# Autodesk Inventor assembly: CC
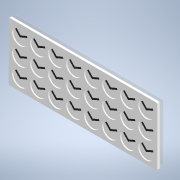
[picture p0: Inventor's stored thumbnail of the model, 180x180]
Saved by Autodesk Inventor 2020 (Build 240168000, 168)
## iProperties
Created: 2019-07-03
Part Number: CC
Document SubType Name: Assembly
Designer: andwh
Author: andwh
## Documents named in this file (6)
- C:\Users\andwh\Documents\Projects\Clock Clock\CC.iam
- C:\Users\andwh\Documents\Projects\Clock Clock\CC-topPlate.ipt
- C:\Users\andwh\Documents\Projects\Clock Clock\Parts\94459A140_BRASS HEAT-SET INSERT FOR PLASTIC.ipt
- C:\Users\andwh\Documents\Projects\Clock Clock\PCB\Clock Board V2\Clock Board V2.iam
- C:\Users\andwh\Documents\Projects\Clock Clock\CC-bottomStand.ipt
- C:\Users\andwh\Documents\Projects\Clock Clock\CC-bottomPlate.ipt
## Components (126 placed, 5 different names)
1. CC-topPlate:1 — Insert:1, Insert:2, Mate:1
2. CC-bottomPlate:1 — Insert:5, Insert:6
3. Clock Board V2:1 [sub-assembly] — Insert:2, Mate:1
4. Clock Board V2:2 [sub-assembly]
5. Clock Board V2:3 [sub-assembly]
6. Clock Board V2:4 [sub-assembly]
7. Clock Board V2:5 [sub-assembly]
8. Clock Board V2:6 [sub-assembly]
9. Clock Board V2:7 [sub-assembly]
10. Clock Board V2:8 [sub-assembly]
11. Clock Board V2:9 [sub-assembly]
12. Clock Board V2:10 [sub-assembly]
13. Clock Board V2:11 [sub-assembly]
14. Clock Board V2:12 [sub-assembly]
15. Clock Board V2:13 [sub-assembly]
16. Clock Board V2:14 [sub-assembly]
17. Clock Board V2:15 [sub-assembly]
18. Clock Board V2:16 [sub-assembly]
19. Clock Board V2:17 [sub-assembly]
20. Clock Board V2:18 [sub-assembly]
21. Clock Board V2:19 [sub-assembly] — Insert:4
22. Clock Board V2:20 [sub-assembly]
23. Clock Board V2:21 [sub-assembly]
24. Clock Board V2:22 [sub-assembly] — Insert:3
25. Clock Board V2:23 [sub-assembly]
26. Clock Board V2:24 [sub-assembly] — Insert:5, Insert:6
27. CC-bottomStand:1 — Insert:3, Insert:4
28. CC-bottomStand:2
29. CC-bottomStand:3
30. CC-bottomStand:4
31. 94459A140_BRASS HEAT-SET INSERT FOR PLASTIC:1 — Insert:1
32. 94459A140_BRASS HEAT-SET INSERT FOR PLASTIC:2
33. 94459A140_BRASS HEAT-SET INSERT FOR PLASTIC:3
34. 94459A140_BRASS HEAT-SET INSERT FOR PLASTIC:4
35. 94459A140_BRASS HEAT-SET INSERT FOR PLASTIC:5
36. 94459A140_BRASS HEAT-SET INSERT FOR PLASTIC:6
37. 94459A140_BRASS HEAT-SET INSERT FOR PLASTIC:7
38. 94459A140_BRASS HEAT-SET INSERT FOR PLASTIC:8
39. 94459A140_BRASS HEAT-SET INSERT FOR PLASTIC:9
40. 94459A140_BRASS HEAT-SET INSERT FOR PLASTIC:10
41. 94459A140_BRASS HEAT-SET INSERT FOR PLASTIC:11
42. 94459A140_BRASS HEAT-SET INSERT FOR PLASTIC:12
43. 94459A140_BRASS HEAT-SET INSERT FOR PLASTIC:13
44. 94459A140_BRASS HEAT-SET INSERT FOR PLASTIC:14
45. 94459A140_BRASS HEAT-SET INSERT FOR PLASTIC:15
46. 94459A140_BRASS HEAT-SET INSERT FOR PLASTIC:16
47. 94459A140_BRASS HEAT-SET INSERT FOR PLASTIC:17
48. 94459A140_BRASS HEAT-SET INSERT FOR PLASTIC:18
49. 94459A140_BRASS HEAT-SET INSERT FOR PLASTIC:19
50. 94459A140_BRASS HEAT-SET INSERT FOR PLASTIC:20
51. 94459A140_BRASS HEAT-SET INSERT FOR PLASTIC:21
52. 94459A140_BRASS HEAT-SET INSERT FOR PLASTIC:22
53. 94459A140_BRASS HEAT-SET INSERT FOR PLASTIC:23
54. 94459A140_BRASS HEAT-SET INSERT FOR PLASTIC:24
55. 94459A140_BRASS HEAT-SET INSERT FOR PLASTIC:25
56. 94459A140_BRASS HEAT-SET INSERT FOR PLASTIC:26
57. 94459A140_BRASS HEAT-SET INSERT FOR PLASTIC:27
58. 94459A140_BRASS HEAT-SET INSERT FOR PLASTIC:28
59. 94459A140_BRASS HEAT-SET INSERT FOR PLASTIC:29
60. 94459A140_BRASS HEAT-SET INSERT FOR PLASTIC:30
61. 94459A140_BRASS HEAT-SET INSERT FOR PLASTIC:31
62. 94459A140_BRASS HEAT-SET INSERT FOR PLASTIC:32
63. 94459A140_BRASS HEAT-SET INSERT FOR PLASTIC:33
64. 94459A140_BRASS HEAT-SET INSERT FOR PLASTIC:34
65. 94459A140_BRASS HEAT-SET INSERT FOR PLASTIC:35
66. 94459A140_BRASS HEAT-SET INSERT FOR PLASTIC:36
67. 94459A140_BRASS HEAT-SET INSERT FOR PLASTIC:37
68. 94459A140_BRASS HEAT-SET INSERT FOR PLASTIC:38
69. 94459A140_BRASS HEAT-SET INSERT FOR PLASTIC:39
70. 94459A140_BRASS HEAT-SET INSERT FOR PLASTIC:40
71. 94459A140_BRASS HEAT-SET INSERT FOR PLASTIC:41
72. 94459A140_BRASS HEAT-SET INSERT FOR PLASTIC:42
73. 94459A140_BRASS HEAT-SET INSERT FOR PLASTIC:43
74. 94459A140_BRASS HEAT-SET INSERT FOR PLASTIC:44
75. 94459A140_BRASS HEAT-SET INSERT FOR PLASTIC:45
76. 94459A140_BRASS HEAT-SET INSERT FOR PLASTIC:46
77. 94459A140_BRASS HEAT-SET INSERT FOR PLASTIC:47
78. 94459A140_BRASS HEAT-SET INSERT FOR PLASTIC:48
79. 94459A140_BRASS HEAT-SET INSERT FOR PLASTIC:49
80. 94459A140_BRASS HEAT-SET INSERT FOR PLASTIC:50
81. 94459A140_BRASS HEAT-SET INSERT FOR PLASTIC:51
82. 94459A140_BRASS HEAT-SET INSERT FOR PLASTIC:52
83. 94459A140_BRASS HEAT-SET INSERT FOR PLASTIC:53
84. 94459A140_BRASS HEAT-SET INSERT FOR PLASTIC:54
85. 94459A140_BRASS HEAT-SET INSERT FOR PLASTIC:55
86. 94459A140_BRASS HEAT-SET INSERT FOR PLASTIC:56
87. 94459A140_BRASS HEAT-SET INSERT FOR PLASTIC:57
88. 94459A140_BRASS HEAT-SET INSERT FOR PLASTIC:58
89. 94459A140_BRASS HEAT-SET INSERT FOR PLASTIC:59
90. 94459A140_BRASS HEAT-SET INSERT FOR PLASTIC:60
91. 94459A140_BRASS HEAT-SET INSERT FOR PLASTIC:61
92. 94459A140_BRASS HEAT-SET INSERT FOR PLASTIC:62
93. 94459A140_BRASS HEAT-SET INSERT FOR PLASTIC:63
94. 94459A140_BRASS HEAT-SET INSERT FOR PLASTIC:64
95. 94459A140_BRASS HEAT-SET INSERT FOR PLASTIC:65
96. 94459A140_BRASS HEAT-SET INSERT FOR PLASTIC:66
97. 94459A140_BRASS HEAT-SET INSERT FOR PLASTIC:67
98. 94459A140_BRASS HEAT-SET INSERT FOR PLASTIC:68
99. 94459A140_BRASS HEAT-SET INSERT FOR PLASTIC:69
100. 94459A140_BRASS HEAT-SET INSERT FOR PLASTIC:70
101. 94459A140_BRASS HEAT-SET INSERT FOR PLASTIC:71
102. 94459A140_BRASS HEAT-SET INSERT FOR PLASTIC:72
103. 94459A140_BRASS HEAT-SET INSERT FOR PLASTIC:73
104. 94459A140_BRASS HEAT-SET INSERT FOR PLASTIC:74
105. 94459A140_BRASS HEAT-SET INSERT FOR PLASTIC:75
106. 94459A140_BRASS HEAT-SET INSERT FOR PLASTIC:76
107. 94459A140_BRASS HEAT-SET INSERT FOR PLASTIC:77
108. 94459A140_BRASS HEAT-SET INSERT FOR PLASTIC:78
109. 94459A140_BRASS HEAT-SET INSERT FOR PLASTIC:79
110. 94459A140_BRASS HEAT-SET INSERT FOR PLASTIC:80
111. 94459A140_BRASS HEAT-SET INSERT FOR PLASTIC:81
112. 94459A140_BRASS HEAT-SET INSERT FOR PLASTIC:82
113. 94459A140_BRASS HEAT-SET INSERT FOR PLASTIC:83
114. 94459A140_BRASS HEAT-SET INSERT FOR PLASTIC:84
115. 94459A140_BRASS HEAT-SET INSERT FOR PLASTIC:85
116. 94459A140_BRASS HEAT-SET INSERT FOR PLASTIC:86
117. 94459A140_BRASS HEAT-SET INSERT FOR PLASTIC:87
118. 94459A140_BRASS HEAT-SET INSERT FOR PLASTIC:88
119. 94459A140_BRASS HEAT-SET INSERT FOR PLASTIC:89
120. 94459A140_BRASS HEAT-SET INSERT FOR PLASTIC:90
121. 94459A140_BRASS HEAT-SET INSERT FOR PLASTIC:91
122. 94459A140_BRASS HEAT-SET INSERT FOR PLASTIC:92
123. 94459A140_BRASS HEAT-SET INSERT FOR PLASTIC:93
124. 94459A140_BRASS HEAT-SET INSERT FOR PLASTIC:94
125. 94459A140_BRASS HEAT-SET INSERT FOR PLASTIC:95
126. 94459A140_BRASS HEAT-SET INSERT FOR PLASTIC:96
## Component patterns: (24 elements, first: Clock Board V2:1), (4 elements, first: CC-bottomStand:1), (4 elements, first: 94459A140_BRASS HEAT-SET INSERT FOR PLASTIC:1), Component Pattern 1:2 (4 elements), Component Pattern 1:3 (4 elements), Component Pattern 1:4 (4 elements), Component Pattern 1:5 (4 elements), Component Pattern 1:6 (4 elements), Component Pattern 1:7 (4 elements), Component Pattern 1:8 (4 elements), Component Pattern 1:9 (4 elements), Component Pattern 1:10 (4 elements), Component Pattern 1:11 (4 elements), Component Pattern 1:12 (4 elements), Component Pattern 1:13 (4 elements), Component Pattern 1:14 (4 elements), Component Pattern 1:15 (4 elements), Component Pattern 1:16 (4 elements), Component Pattern 1:17 (4 elements), Component Pattern 1:18 (4 elements), Component Pattern 1:19 (4 elements), Component Pattern 1:20 (4 elements), Component Pattern 1:21 (4 elements), Component Pattern 1:22 (4 elements), Component Pattern 1:23 (4 elements), Component Pattern 1:24 (4 elements)
## Relationships (7: Insert 6, Mate 1)
- Insert:1: CC-topPlate:1 ↔ 94459A140_BRASS HEAT-SET INSERT FOR PLASTIC:1
- Insert:2: CC-topPlate:1 ↔ Clock Board V2:1
- Mate:1: CC-topPlate:1 ↔ Clock Board V2:1
- Insert:3: Clock Board V2:22 ↔ CC-bottomStand:1
- Insert:4: Clock Board V2:19 ↔ CC-bottomStand:1
- Insert:5: CC-bottomPlate:1 ↔ Clock Board V2:24
- Insert:6: CC-bottomPlate:1 ↔ Clock Board V2:24
